# Autodesk Inventor assembly: QuicrunESCAssembly
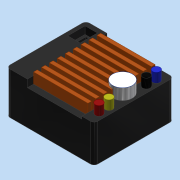
[picture p0: Inventor's stored thumbnail of the model, 180x180]
Saved by Autodesk Inventor 2017 (Build 210142000, 142)
## iProperties
Created: 2017-01-26
Part Number: QuicrunESCAssembly
Document SubType Name: Assembly
Designer: techn
Mass: 45.3592 g
Surface Area: 123.467 cm^2
Volume: 11.4828 cm^3
Author: techn
## Documents named in this file (8)
- G:\Projects\Submarine\Submarine-project\CAD\midships\ElectronicsSection\QUICRUN ESC\QuicrunESCAssembly.iam
- G:\Projects\Submarine\Submarine-project\CAD\midships\ElectronicsSection\QUICRUN ESC\body.ipt
- G:\Projects\Submarine\Submarine-project\CAD\midships\ElectronicsSection\QUICRUN ESC\Cap.ipt
- G:\Projects\Submarine\Submarine-project\CAD\midships\ElectronicsSection\QUICRUN ESC\Heatsink.ipt
- G:\Projects\Submarine\Submarine-project\CAD\midships\ElectronicsSection\QUICRUN ESC\BlackWire.ipt
- G:\Projects\Submarine\Submarine-project\CAD\midships\ElectronicsSection\QUICRUN ESC\BlueWire.ipt
- G:\Projects\Submarine\Submarine-project\CAD\midships\ElectronicsSection\QUICRUN ESC\RedWire.ipt
- G:\Projects\Submarine\Submarine-project\CAD\midships\ElectronicsSection\QUICRUN ESC\YellowWire.ipt
## Components (7 placed, 7 different names)
1. body:1 — Mate:1, Mate:2, Mate:3, Flush:1, Mate:4, Mate:5, Mate:6, Mate:7, Flush:6
2. Cap:1 — Mate:1, Flush:2
3. Heatsink:1 — Mate:2, Mate:3, Flush:1, Flush:2
4. BlackWire:1 — Mate:5, Flush:3, Flush:4
5. BlueWire:1 — Mate:4, Flush:3, Flush:6
6. RedWire:1 — Mate:7, Flush:5
7. YellowWire:1 — Mate:6, Flush:4, Flush:5
## Relationships (13: Mate 7, Flush 6)
- Mate:1: body:1 ↔ Cap:1
- Mate:2: body:1 ↔ Heatsink:1
- Mate:3: body:1 ↔ Heatsink:1
- Flush:1 (-1.27 mm): body:1 ↔ Heatsink:1
- Flush:2 (-1.27 mm): Cap:1 ↔ Heatsink:1
- Mate:4: body:1 ↔ BlueWire:1
- Mate:5: body:1 ↔ BlackWire:1
- Mate:6: body:1 ↔ YellowWire:1
- Mate:7: body:1 ↔ RedWire:1
- Flush:3: BlackWire:1 ↔ BlueWire:1
- Flush:4: BlackWire:1 ↔ YellowWire:1
- Flush:5: RedWire:1 ↔ YellowWire:1
- Flush:6 (-3.81 mm): body:1 ↔ BlueWire:1
